# Autodesk Inventor assembly: BoltWasher3x8
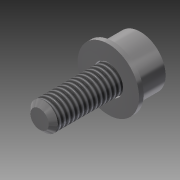
[picture p0: Inventor's stored thumbnail of the model, 180x180]
Saved by Autodesk Inventor 2015 SP1 (Build 190203100, 203)
## iProperties
Category: Hardware
Created: 2015-01-21
Part Number: BoltWasher3x8
Document SubType Name: Assembly
Designer: Jack
Mass: 1.03755 g
Surface Area: 2.58965 cm^2
Volume: 0.129558 cm^3
Density: 8.0084 g/cm^3
Vendor: Misumi
Author: Jack
Title: Bolt + Washer 3x8
## Documents named in this file (3)
- C:\Users\Jack\ownCloud\Projects\CoreXY\InventorModel\Hardware\BoltWashers\BoltWasher3\BoltWasher3x8.iam
- C:\Users\Jack\ownCloud\Projects\CoreXY\InventorModel\Hardware\Wahsers\M3Washer.ipt
- C:\Users\Jack\ownCloud\Projects\CoreXY\InventorModel\Hardware\Bolts\SHCS\SHCS3\SHCS3x8.ipt
## Components (2 placed, 2 different names)
1. M3Washer:1 — Mate:1, Mate:2
2. SHCS3x8:1 — Mate:1, Mate:2
## Relationships (2: Mate 2)
- Mate:1: M3Washer:1 ↔ SHCS3x8:1
- Mate:2: M3Washer:1 ↔ SHCS3x8:1
